# Autodesk Inventor assembly: 機体
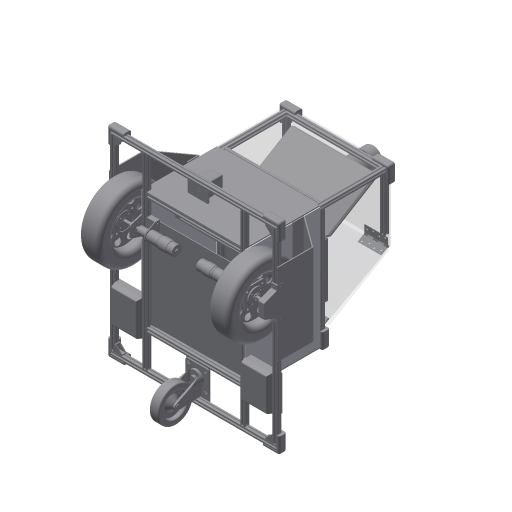
[picture p0: Inventor's stored thumbnail of the model, 512x512]
Saved by Autodesk Inventor 2023 (Build 270158000, 158)
## iProperties
Part Number: 機体
Material: 一般
Document SubType Name: Assembly
Designer: highs
Author: highs
## Documents named in this file (25)
- C:\Users\shunyahara\Downloads\newnaviton-20230713T030115Z-001\newnaviton\Navitoon\機体.iam
- C:\Users\shunyahara\Downloads\newnaviton-20230713T030115Z-001\newnaviton\Navitoon\フレーム.iam
- C:\Users\shunyahara\Downloads\newnaviton-20230713T030115Z-001\newnaviton\Navitoon\車輪部分.iam
- C:\Users\shunyahara\Downloads\newnaviton-20230713T030115Z-001\newnaviton\Navitoon\自由輪部分.iam
- C:\Users\shunyahara\Downloads\newnaviton-20230713T030115Z-001\newnaviton\Navitoon\ライダーマウント.ipt
- C:\Users\shunyahara\Downloads\newnaviton-20230713T030115Z-001\newnaviton\Navitoon\PCパーツ1.ipt
- C:\Users\shunyahara\Downloads\newnaviton-20230713T030115Z-001\newnaviton\Navitoon\PCパーツ2.ipt
- C:\Users\shunyahara\Downloads\newnaviton-20230713T030115Z-001\newnaviton\Navitoon\回路スペース.ipt
- C:\Users\shunyahara\Downloads\newnaviton-20230713T030115Z-001\newnaviton\Navitoon\防水1.ipt
- C:\Users\shunyahara\Downloads\newnaviton-20230713T030115Z-001\newnaviton\Navitoon\防水3.ipt
- C:\Users\shunyahara\Downloads\newnaviton-20230713T030115Z-001\newnaviton\Navitoon\防水2.ipt
- C:\Users\shunyahara\Downloads\newnaviton-20230713T030115Z-001\newnaviton\Navitoon\蝶番1.ipt
- C:\Users\shunyahara\Downloads\newnaviton-20230713T030115Z-001\newnaviton\Navitoon\蝶番2.ipt
- C:\Users\shunyahara\Downloads\newnaviton-20230713T030115Z-001\newnaviton\Navitoon\防水4.ipt
- C:\Users\shunyahara\Downloads\newnaviton-20230713T030115Z-001\newnaviton\Navitoon\防水p1.ipt
- C:\Users\shunyahara\Downloads\newnaviton-20230713T030115Z-001\newnaviton\Navitoon\防水5.ipt
- C:\Users\shunyahara\Downloads\newnaviton-20230713T030115Z-001\newnaviton\Navitoon\防水p2.ipt
- C:\Users\shunyahara\Downloads\newnaviton-20230713T030115Z-001\newnaviton\Navitoon\防水p3.ipt
- C:\Users\shunyahara\Downloads\newnaviton-20230713T030115Z-001\newnaviton\Navitoon\防水p4.ipt
- C:\Users\shunyahara\Downloads\newnaviton-20230713T030115Z-001\newnaviton\Navitoon\クッション.ipt
- C:\Users\shunyahara\Downloads\newnaviton-20230713T030115Z-001\newnaviton\Navitoon\回路スペース2.ipt
- C:\Users\shunyahara\Downloads\newnaviton-20230713T030115Z-001\newnaviton\Navitoon\タイヤカバー.ipt
- C:\Users\shunyahara\Downloads\newnaviton-20230713T030115Z-001\newnaviton\Navitoon\おもり.ipt
- C:\Users\shunyahara\Downloads\newnaviton-20230713T030115Z-001\newnaviton\Navitoon\raida- .ipt
- C:\Users\shunyahara\Downloads\newnaviton-20230713T030115Z-001\newnaviton\Navitoon\hdl32e.ipt
## Components (39 placed, 24 different names)
1. フレーム:1 [sub-assembly] — メイト:1, フラッシュ:1, フラッシュ:2, メイト:2, フラッシュ:4, メイト:3, フラッシュ:5, フラッシュ:10, メイト:12, フラッシュ:21, メイト:25, メイト:26, フラッシュ:22, フラッシュ:23, フラッシュ:24, フラッシュ:25, メイト:27, フラッシュ:26, フラッシュ:27, メイト:40, フラッシュ:30, メイト:42, フラッシュ:44, フラッシュ:45, メイト:43, メイト:44, フラッシュ:46, フラッシュ:47, メイト:45, フラッシュ:50, メイト:48, フラッシュ:51, フラッシュ:52, フラッシュ:55, メイト:49, フラッシュ:56, フラッシュ:57, メイト:50, メイト:57, メイト:62, メイト:63, フラッシュ:60, フラッシュ:61, メイト:64, メイト:65, メイト:66, メイト:67, メイト:68, メイト:69, メイト:70, メイト:71, メイト:72, メイト:73, メイト:74, メイト:75, フラッシュ:62, フラッシュ:64, メイト:78, フラッシュ:66, メイト:79, フラッシュ:68, メイト:81, フラッシュ:69, メイト:82
2. 車輪部分:1 [sub-assembly] — フラッシュ:2, メイト:2, フラッシュ:10, フラッシュ:11
3. 車輪部分:2 [sub-assembly] — メイト:1, フラッシュ:1, フラッシュ:11
4. 自由輪部分:1 [sub-assembly] — メイト:3, フラッシュ:5, フラッシュ:21
5. PCパーツ1:2 — メイト:13, メイト:14, メイト:47, 角度:1
6. 回路スペース:1 — メイト:12
7. PCパーツ2:2 — メイト:13, メイト:14
8. 防水1:1 — メイト:25, フラッシュ:22, フラッシュ:23, フラッシュ:49
9. 防水1:2 — メイト:26, フラッシュ:24, フラッシュ:25, フラッシュ:48, メイト:85
10. 防水3:1 — メイト:36, メイト:37, メイト:38, メイト:39
11. 防水2:1 — メイト:27, フラッシュ:26, フラッシュ:27, メイト:30, メイト:31, メイト:32, メイト:33, メイト:34, メイト:35, メイト:41, メイト:51, メイト:52, メイト:53, メイト:54, メイト:55, メイト:56, メイト:84
12. 蝶番1:1 — メイト:28, フラッシュ:28, メイト:36, メイト:37, メイト:38
13. 蝶番2:1 — メイト:28, フラッシュ:28, メイト:31, メイト:32, メイト:33
14. 蝶番1:2 — メイト:29, フラッシュ:29, メイト:39
15. 蝶番2:2 — メイト:29, フラッシュ:29, メイト:30, メイト:34, メイト:35
16. 防水4:1 — メイト:40, フラッシュ:30, メイト:41, フラッシュ:72
17. 防水p1:1 — メイト:42, フラッシュ:44, フラッシュ:45, メイト:47, 角度:1, フラッシュ:59, メイト:58
18. 防水5:1 — メイト:43, フラッシュ:46, フラッシュ:49
19. 防水5:2 — メイト:44, フラッシュ:47, フラッシュ:48
20. 防水p2:1 — メイト:45, フラッシュ:50, フラッシュ:55, メイト:61, メイト:77
21. 防水p2:2 — メイト:48, フラッシュ:51, フラッシュ:52, フラッシュ:58, メイト:76
22. 防水p3:2 — メイト:49, フラッシュ:56, フラッシュ:57, フラッシュ:63, フラッシュ:65
23. 防水p4:1 — フラッシュ:58, メイト:50, フラッシュ:59, メイト:59, メイト:60
24. クッション:1 — メイト:54, メイト:55, メイト:56
25. クッション:2 — メイト:51, メイト:52, メイト:53
26. クッション:3 — メイト:60, メイト:61, メイト:62
27. クッション:4 — メイト:57, メイト:58, メイト:59
28. 回路スペース2:1 — メイト:63, フラッシュ:60, フラッシュ:61
29. クッション:5 — メイト:64, メイト:71, メイト:72
30. クッション:6 — メイト:65, メイト:74, メイト:75
31. クッション:7 — メイト:66, メイト:68, メイト:69
32. クッション:8 — メイト:67, メイト:70, メイト:73
33. タイヤカバー:1 — メイト:76, フラッシュ:62, フラッシュ:63
34. タイヤカバー:2 — メイト:77, フラッシュ:64, フラッシュ:65
35. おもり:1 — メイト:78, フラッシュ:66, フラッシュ:67
36. おもり:2 — メイト:79, フラッシュ:67, フラッシュ:68
37. ライダーマウント:5 — メイト:81, フラッシュ:69, メイト:82, メイト:83, フラッシュ:70, フラッシュ:71
38. raida- :1 — メイト:83, フラッシュ:70, フラッシュ:71
39. hdl32e:1 — メイト:84, メイト:85, フラッシュ:72
## Relationships (109: Mate 65, Flush 43, Angle 1)
- メイト:1 [Mate]: フレーム:1 ↔ 車輪部分:2
- フラッシュ:1 [Flush]: フレーム:1 ↔ 車輪部分:2
- フラッシュ:2 [Flush]: フレーム:1 ↔ 車輪部分:1
- メイト:2 [Mate]: フレーム:1 ↔ 車輪部分:1
- フラッシュ:4 [Flush] (172 mm): フレーム:1
- メイト:3 [Mate]: フレーム:1 ↔ 自由輪部分:1
- フラッシュ:5 [Flush]: フレーム:1 ↔ 自由輪部分:1
- フラッシュ:10 [Flush] (230 mm): フレーム:1 ↔ 車輪部分:1
- フラッシュ:11 [Flush]: 車輪部分:1 ↔ 車輪部分:2
- メイト:12 [Mate]: フレーム:1 ↔ 回路スペース:1
- メイト:13 [Mate]: PCパーツ1:2 ↔ PCパーツ2:2
- メイト:14 [Mate]: PCパーツ1:2 ↔ PCパーツ2:2
- フラッシュ:21 [Flush] (-170 mm): フレーム:1 ↔ 自由輪部分:1
- メイト:25 [Mate]: フレーム:1 ↔ 防水1:1
- メイト:26 [Mate]: フレーム:1 ↔ 防水1:2
- フラッシュ:22 [Flush]: フレーム:1 ↔ 防水1:1
- フラッシュ:23 [Flush]: フレーム:1 ↔ 防水1:1
- フラッシュ:24 [Flush]: フレーム:1 ↔ 防水1:2
- フラッシュ:25 [Flush]: フレーム:1 ↔ 防水1:2
- メイト:27 [Mate]: フレーム:1 ↔ 防水2:1
- フラッシュ:26 [Flush] (6 mm): フレーム:1 ↔ 防水2:1
- フラッシュ:27 [Flush] (5 mm): フレーム:1 ↔ 防水2:1
- メイト:28 [Mate]: 蝶番1:1 ↔ 蝶番2:1
- フラッシュ:28 [Flush]: 蝶番1:1 ↔ 蝶番2:1
- メイト:29 [Mate]: 蝶番1:2 ↔ 蝶番2:2
- フラッシュ:29 [Flush]: 蝶番1:2 ↔ 蝶番2:2
- メイト:30 [Mate]: 防水2:1 ↔ 蝶番2:2
- メイト:31 [Mate]: 防水2:1 ↔ 蝶番2:1
- メイト:32 [Mate]: 防水2:1 ↔ 蝶番2:1
- メイト:33 [Mate]: 防水2:1 ↔ 蝶番2:1
- メイト:34 [Mate]: 防水2:1 ↔ 蝶番2:2
- メイト:35 [Mate]: 防水2:1 ↔ 蝶番2:2
- メイト:36 [Mate]: 防水3:1 ↔ 蝶番1:1
- メイト:37 [Mate]: 防水3:1 ↔ 蝶番1:1
- メイト:38 [Mate]: 防水3:1 ↔ 蝶番1:1
- メイト:39 [Mate]: 防水3:1 ↔ 蝶番1:2
- メイト:40 [Mate]: フレーム:1 ↔ 防水4:1
- フラッシュ:30 [Flush] (-5 mm): フレーム:1 ↔ 防水4:1
- メイト:41 [Mate]: 防水2:1 ↔ 防水4:1
- メイト:42 [Mate]: フレーム:1 ↔ 防水p1:1
- フラッシュ:44 [Flush]: フレーム:1 ↔ 防水p1:1
- フラッシュ:45 [Flush]: フレーム:1 ↔ 防水p1:1
- メイト:43 [Mate]: フレーム:1 ↔ 防水5:1
- メイト:44 [Mate]: フレーム:1 ↔ 防水5:2
- フラッシュ:46 [Flush]: フレーム:1 ↔ 防水5:1
- フラッシュ:47 [Flush]: フレーム:1 ↔ 防水5:2
- フラッシュ:48 [Flush]: 防水1:2 ↔ 防水5:2
- フラッシュ:49 [Flush]: 防水1:1 ↔ 防水5:1
- メイト:45 [Mate]: フレーム:1 ↔ 防水p2:1
- フラッシュ:50 [Flush]: フレーム:1 ↔ 防水p2:1
- メイト:47 [Mate]: PCパーツ1:2 ↔ 防水p1:1
- 角度:1 [Angle] (0 deg): PCパーツ1:2 ↔ 防水p1:1
- メイト:48 [Mate]: フレーム:1 ↔ 防水p2:2
- フラッシュ:51 [Flush]: フレーム:1 ↔ 防水p2:2
- フラッシュ:52 [Flush]: フレーム:1 ↔ 防水p2:2
- フラッシュ:55 [Flush]: フレーム:1 ↔ 防水p2:1
- メイト:49 [Mate]: フレーム:1 ↔ 防水p3:2
- フラッシュ:56 [Flush]: フレーム:1 ↔ 防水p3:2
- フラッシュ:57 [Flush]: フレーム:1 ↔ 防水p3:2
- フラッシュ:58 [Flush]: 防水p2:2 ↔ 防水p4:1
- メイト:50 [Mate]: フレーム:1 ↔ 防水p4:1
- フラッシュ:59 [Flush]: 防水p1:1 ↔ 防水p4:1
- メイト:51 [Mate]: 防水2:1 ↔ クッション:2
- メイト:52 [Mate]: 防水2:1 ↔ クッション:2
- メイト:53 [Mate]: 防水2:1 ↔ クッション:2
- メイト:54 [Mate]: 防水2:1 ↔ クッション:1
- メイト:55 [Mate]: 防水2:1 ↔ クッション:1
- メイト:56 [Mate]: 防水2:1 ↔ クッション:1
- メイト:57 [Mate]: フレーム:1 ↔ クッション:4
- メイト:58 [Mate]: 防水p1:1 ↔ クッション:4
- メイト:59 [Mate]: 防水p4:1 ↔ クッション:4
- メイト:60 [Mate]: 防水p4:1 ↔ クッション:3
- メイト:61 [Mate]: 防水p2:1 ↔ クッション:3
- メイト:62 [Mate]: フレーム:1 ↔ クッション:3
- メイト:63 [Mate]: フレーム:1 ↔ 回路スペース2:1
- フラッシュ:60 [Flush]: フレーム:1 ↔ 回路スペース2:1
- フラッシュ:61 [Flush]: フレーム:1 ↔ 回路スペース2:1
- メイト:64 [Mate]: フレーム:1 ↔ クッション:5
- メイト:65 [Mate]: フレーム:1 ↔ クッション:6
- メイト:66 [Mate]: フレーム:1 ↔ クッション:7
- メイト:67 [Mate]: フレーム:1 ↔ クッション:8
- メイト:68 [Mate]: フレーム:1 ↔ クッション:7
- メイト:69 [Mate]: フレーム:1 ↔ クッション:7
- メイト:70 [Mate]: フレーム:1 ↔ クッション:8
- メイト:71 [Mate]: フレーム:1 ↔ クッション:5
- メイト:72 [Mate]: フレーム:1 ↔ クッション:5
- メイト:73 [Mate]: フレーム:1 ↔ クッション:8
- メイト:74 [Mate]: フレーム:1 ↔ クッション:6
- メイト:75 [Mate]: フレーム:1 ↔ クッション:6
- メイト:76 [Mate]: 防水p2:2 ↔ タイヤカバー:1
- フラッシュ:62 [Flush]: フレーム:1 ↔ タイヤカバー:1
- フラッシュ:63 [Flush]: 防水p3:2 ↔ タイヤカバー:1
- メイト:77 [Mate]: 防水p2:1 ↔ タイヤカバー:2
- フラッシュ:64 [Flush]: フレーム:1 ↔ タイヤカバー:2
- フラッシュ:65 [Flush]: 防水p3:2 ↔ タイヤカバー:2
- メイト:78 [Mate]: フレーム:1 ↔ おもり:1
- フラッシュ:66 [Flush]: フレーム:1 ↔ おもり:1
- メイト:79 [Mate]: フレーム:1 ↔ おもり:2
- フラッシュ:67 [Flush]: おもり:1 ↔ おもり:2
- フラッシュ:68 [Flush]: フレーム:1 ↔ おもり:2
- メイト:81 [Mate]: フレーム:1 ↔ ライダーマウント:5
- フラッシュ:69 [Flush]: フレーム:1 ↔ ライダーマウント:5
- メイト:82 [Mate] (293 mm): フレーム:1 ↔ ライダーマウント:5
- メイト:83 [Mate]: ライダーマウント:5 ↔ raida- :1
- フラッシュ:70 [Flush] (15 mm): ライダーマウント:5 ↔ raida- :1
- フラッシュ:71 [Flush] (-25 mm): ライダーマウント:5 ↔ raida- :1
- メイト:84 [Mate]: 防水2:1 ↔ hdl32e:1
- メイト:85 [Mate] (-222 mm): 防水1:2 ↔ hdl32e:1
- フラッシュ:72 [Flush] (120 mm): 防水4:1 ↔ hdl32e:1
